# Autodesk Inventor assembly: RoboCinWheel_simplified
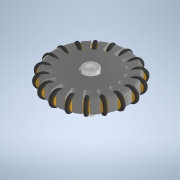
[picture p0: Inventor's stored thumbnail of the model, 180x180]
Saved by Autodesk Inventor 2021 (Build 250183000, 183)
## iProperties
Created: 2022-09-21
Part Number: RoboCinWheel_simplified
Document SubType Name: Assembly
Designer: victo
Author: victo
## Documents named in this file (4)
- C:\Users\victo\Documents\MATLAB\CAD\Inventor\first_floor\Wheel\RoboCinWheel_simplified.iam
- C:\Users\victo\Documents\MATLAB\CAD\Inventor\first_floor\Wheel\wheel_simplified2.ipt
- C:\Users\victo\Documents\MATLAB\CAD\Inventor\first_floor\Wheel\gear_z60_26106000_simplified.ipt
- C:\Users\victo\Documents\MATLAB\CAD\Inventor\first_floor\Wheel\Roller.iam
## Components (20 placed, 3 different names)
1. wheel_simplified2:1 — Cylindrical:1, Cylindrical:2, Cylindrical:3, Cylindrical:4, Cylindrical:5, Cylindrical:6, Cylindrical:7, Cylindrical:8, Cylindrical:9, Cylindrical:10, Cylindrical:11, Cylindrical:12, Cylindrical:13, Cylindrical:14, Cylindrical:15, Cylindrical:16, Cylindrical:17, Cylindrical:18, Rigid:1
2. gear_z60_26106000_simplified:1 — Rigid:1
3. Roller:1 [sub-assembly] — Cylindrical:3
4. Roller:2 [sub-assembly] — Cylindrical:1
5. Roller:3 [sub-assembly] — Cylindrical:2
6. Roller:4 [sub-assembly] — Cylindrical:4
7. Roller:5 [sub-assembly] — Cylindrical:5
8. Roller:6 [sub-assembly] — Cylindrical:6
9. Roller:7 [sub-assembly] — Cylindrical:7
10. Roller:8 [sub-assembly] — Cylindrical:8
11. Roller:9 [sub-assembly] — Cylindrical:9
12. Roller:10 [sub-assembly] — Cylindrical:10
13. Roller:11 [sub-assembly] — Cylindrical:11
14. Roller:12 [sub-assembly] — Cylindrical:12
15. Roller:13 [sub-assembly] — Cylindrical:13
16. Roller:14 [sub-assembly] — Cylindrical:14
17. Roller:15 [sub-assembly] — Cylindrical:15
18. Roller:16 [sub-assembly] — Cylindrical:16
19. Roller:17 [sub-assembly] — Cylindrical:17
20. Roller:18 [sub-assembly] — Cylindrical:18
## Relationships (19: CylindricalJoint 18, WeldJoint 1)
- Cylindrical:1: wheel_simplified2:1 ↔ Roller:2
- Cylindrical:2: wheel_simplified2:1 ↔ Roller:3
- Cylindrical:3: wheel_simplified2:1 ↔ Roller:1
- Cylindrical:4: wheel_simplified2:1 ↔ Roller:4
- Cylindrical:5: wheel_simplified2:1 ↔ Roller:5
- Cylindrical:6: wheel_simplified2:1 ↔ Roller:6
- Cylindrical:7: wheel_simplified2:1 ↔ Roller:7
- Cylindrical:8: wheel_simplified2:1 ↔ Roller:8
- Cylindrical:9: wheel_simplified2:1 ↔ Roller:9
- Cylindrical:10: wheel_simplified2:1 ↔ Roller:10
- Cylindrical:11: wheel_simplified2:1 ↔ Roller:11
- Cylindrical:12: wheel_simplified2:1 ↔ Roller:12
- Cylindrical:13: wheel_simplified2:1 ↔ Roller:13
- Cylindrical:14: wheel_simplified2:1 ↔ Roller:14
- Cylindrical:15: wheel_simplified2:1 ↔ Roller:15
- Cylindrical:16: wheel_simplified2:1 ↔ Roller:16
- Cylindrical:17: wheel_simplified2:1 ↔ Roller:17
- Cylindrical:18: wheel_simplified2:1 ↔ Roller:18
- Rigid:1 [WeldJoint]: wheel_simplified2:1 ↔ gear_z60_26106000_simplified:1
